# Autodesk Inventor assembly: Assemb
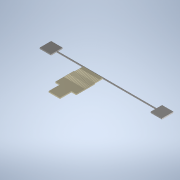
[picture p0: Inventor's stored thumbnail of the model, 180x180]
Saved by Autodesk Inventor 2021 (Build 250183000, 183)
## iProperties
Created: 2023-01-02
Part Number: Assemb
Document SubType Name: Assembly
Designer: omare
Author: omare
## Documents named in this file (4)
- D:\Studying\Engineering\MCTS\Senior 1\First semester\MCT 342 - Introduction to Nano\project\Assemb.iam
- D:\Studying\Engineering\MCTS\Senior 1\First semester\MCT 342 - Introduction to Nano\project\beam.ipt
- D:\Studying\Engineering\MCTS\Senior 1\First semester\MCT 342 - Introduction to Nano\project\bot.ipt
- D:\Studying\Engineering\MCTS\Senior 1\First semester\MCT 342 - Introduction to Nano\project\top.ipt
## Components (3 placed, 3 different names)
1. beam:1 — Mate:1, Mate:2, Mate:3, Mate:4
2. bot:1 — Mate:1, Mate:2, Mate:3, Mate:4, Mate:5, Angle:1, Mate:6, Angle:2, Mate:7
3. top:1 — Mate:5, Angle:1, Mate:6, Angle:2, Mate:8
## Relationships (10: Mate 8, Angle 2)
- Mate:1: beam:1 ↔ bot:1
- Mate:2: beam:1 ↔ bot:1
- Mate:3: beam:1 ↔ bot:1
- Mate:4: beam:1 ↔ bot:1
- Mate:5 (0.0002 mm): bot:1 ↔ top:1
- Angle:1 (0 deg): bot:1 ↔ top:1
- Mate:6 (0.0045 mm): bot:1 ↔ top:1
- Angle:2 (0 deg): bot:1 ↔ top:1
- Mate:7: bot:1
- Mate:8: top:1
